# Autodesk Inventor assembly: FirstAssembly
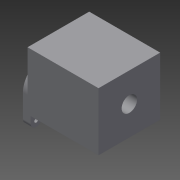
[picture p0: Inventor's stored thumbnail of the model, 180x180]
Saved by Autodesk Inventor 2014 SP1 (Build 180222100, 222)
## iProperties
Created: 2014-03-23
Part Number: FirstAssembly
Document SubType Name: Assembly
Designer: Mark
Author: Mark
## Documents named in this file (3)
- F:\Users\Mark\Documents\inventor\GitHub\FirstAssembly.iam
- F:\Users\Mark\Documents\Inventor\GitHub\BOX.ipt
- F:\Users\Mark\Documents\inventor\GitHub\TEST.ipt
## Components (2 placed, 2 different names)
1. BOX:1 — Rotational:1
2. TEST:1 — Rotational:1
## Relationships (1: RevoluteJoint 1)
- Rotational:1 [RevoluteJoint]: BOX:1 ↔ TEST:1
